# Autodesk Inventor assembly: 739375
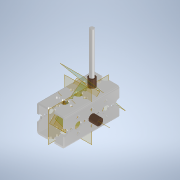
[picture p0: Inventor's stored thumbnail of the model, 180x180]
Saved by Autodesk Inventor 2020.1 (Build 241239000, 239)
## iProperties
Created: 2014-11-26
Part Number: 739375
Document SubType Name: Assembly
Designer: Tetrix
Catalog Web Link: http://www.tetrixrobotics.com/Gears_and_Sprockets/TETRIX_MAX/TETRIX_Worm_Gear_Box
Vendor: Tetrix
Category: Add-on Components
Company: Autodesk Inc.
Author: Autodesk Inc.
## Documents named in this file (10)
- C:\Users\tbloo\Documents\GitHub\AO_Robotics\CAD\Parts Kits\FTC Tetrix KOP Organized (7-24-19)\Gear\Worm Gear\Tetrix_39375.iam
- C:\Users\tbloo\Documents\GitHub\AO_Robotics\CAD\Parts Kits\FTC Tetrix KOP Organized (7-24-19)\Gear\Worm Gear\Tetrix_39375_Shaft.ipt
- C:\Users\tbloo\Documents\GitHub\AO_Robotics\CAD\Parts Kits\FTC Tetrix KOP Organized (7-24-19)\Gear\Worm Gear\Tetrix_39375_Bushing.ipt
- C:\Users\tbloo\Documents\GitHub\AO_Robotics\CAD\Parts Kits\FTC Tetrix KOP Organized (7-24-19)\Gear\Worm Gear\Tetrix_39375_Channel.ipt
- C:\Users\tbloo\Documents\GitHub\AO_Robotics\CAD\Parts Kits\FTC Tetrix KOP Organized (7-24-19)\Gear\Worm Gear\Tetrix_39375_BushingSmall.ipt
- C:\Users\tbloo\Documents\GitHub\AO_Robotics\CAD\Parts Kits\FTC Tetrix KOP Organized (7-24-19)\Gear\Worm Gear\Tetrix_39375_Worm.ipt
- C:\Users\tbloo\Documents\GitHub\AO_Robotics\CAD\Parts Kits\FTC Tetrix KOP Organized (7-24-19)\Gear\Worm Gear\Tetrix_39375_Screw2.ipt
- C:\Users\tbloo\Documents\GitHub\AO_Robotics\CAD\Parts Kits\FTC Tetrix KOP Organized (7-24-19)\Gear\Worm Gear\Tetrix_39375_Screw1.ipt
- C:\Users\tbloo\Documents\GitHub\AO_Robotics\CAD\Parts Kits\FTC Tetrix KOP Organized (7-24-19)\Gear\Worm Gear\Tetrix_39375_Gear.ipt
- C:\Users\tbloo\Documents\GitHub\AO_Robotics\CAD\Parts Kits\FTC Tetrix KOP Organized (7-24-19)\Gear\Worm Gear\Tetrix_39375_Shaft1.ipt
## Components (13 placed, 9 different names)
1. Tetrix_39375_Shaft:1 — Mate:1, Flush:1, Mate:2
2. Tetrix_39375_Bushing:1 — Insert:6, Mate:3
3. Tetrix_39375_Bushing:2 — Insert:4, Flush:1
4. Tetrix_39375_Bushing:3 — Insert:3
5. Tetrix_39375_Channel:1 — Mate:1, Insert:3, Insert:4, Insert:5, Insert:6, Mate:4, Flush:3
6. Tetrix_39375_BushingSmall:1 — Insert:5
7. Tetrix_39375_Worm:1 — Mate:2, Angle:2, Mate:8, Mate:9, Mate:10
8. Tetrix_39375_Screw2:1 — Mate:6, Flush:2
9. Tetrix_39375_Screw2:2 — Mate:5, Flush:2, Symmetry:1
10. Tetrix_39375_Screw1:1 — Mate:9
11. Tetrix_39375_Screw1:2 — Mate:10
12. Tetrix_39375_Gear:1 — Mate:3, Mate:4, Insert:7, Mate:5, Mate:6, Flush:3, Mate:7, Mate:8, Symmetry:1
13. Tetrix_39375_Shaft1:1 — Insert:7
## Relationships (20: Mate 10, Insert 5, Flush 3, Angle 1, Symmetry 1)
- Mate:1: Tetrix_39375_Shaft:1 ↔ Tetrix_39375_Channel:1
- Flush:1: Tetrix_39375_Shaft:1 ↔ Tetrix_39375_Bushing:2
- Insert:3: Tetrix_39375_Bushing:3 ↔ Tetrix_39375_Channel:1
- Mate:2: Tetrix_39375_Shaft:1 ↔ Tetrix_39375_Worm:1
- Insert:4: Tetrix_39375_Bushing:2 ↔ Tetrix_39375_Channel:1
- Insert:5: Tetrix_39375_Channel:1 ↔ Tetrix_39375_BushingSmall:1
- Insert:6: Tetrix_39375_Bushing:1 ↔ Tetrix_39375_Channel:1
- Mate:3: Tetrix_39375_Bushing:1 ↔ Tetrix_39375_Gear:1
- Mate:4: Tetrix_39375_Channel:1 ↔ Tetrix_39375_Gear:1
- Insert:7: Tetrix_39375_Gear:1 ↔ Tetrix_39375_Shaft1:1
- Mate:5: Tetrix_39375_Screw2:2 ↔ Tetrix_39375_Gear:1
- Mate:6: Tetrix_39375_Screw2:1 ↔ Tetrix_39375_Gear:1
- Flush:2: Tetrix_39375_Screw2:1 ↔ Tetrix_39375_Screw2:2
- Flush:3: Tetrix_39375_Channel:1 ↔ Tetrix_39375_Gear:1
- Mate:7: Tetrix_39375_Gear:1
- Angle:2 (90 deg): Tetrix_39375_Worm:1
- Mate:8: Tetrix_39375_Worm:1 ↔ Tetrix_39375_Gear:1
- Symmetry:1: Tetrix_39375_Screw2:2 ↔ Tetrix_39375_Gear:1
- Mate:9: Tetrix_39375_Worm:1 ↔ Tetrix_39375_Screw1:1
- Mate:10: Tetrix_39375_Worm:1 ↔ Tetrix_39375_Screw1:2
